# Autodesk Inventor assembly: insertAssembly-2
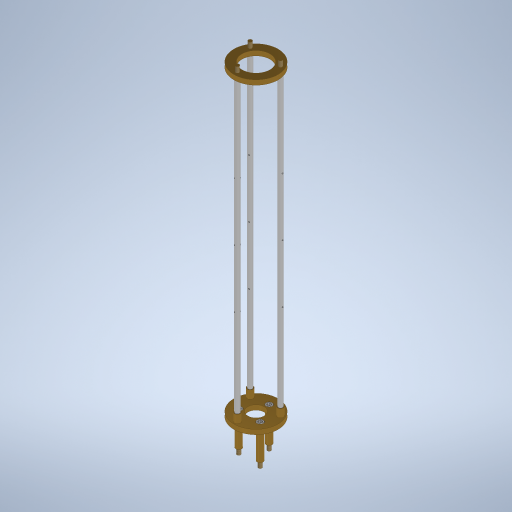
[picture p0: Inventor's stored thumbnail of the model, 512x512]
Saved by Autodesk Inventor 2024 (Build 280153000, 153)
## iProperties
Created: 2023-09-24
Part Number: insertAssembly-2
Document SubType Name: Assembly
Designer: schanen
Author: schanen
## Documents named in this file (6)
- C:\Users\schanen\Documents\Inventor\he4inserts\insertAssembly-2.iam
- C:\Users\schanen\Documents\Inventor\he4inserts\CompositeSupport.iam
- C:\Users\schanen\Documents\Inventor\he4inserts\Insert_flange.ipt
- C:\Users\schanen\Documents\Inventor\he4inserts\Insert_flange_Top.ipt
- C:\Users\schanen\Documents\Inventor\he4inserts\Screw_StainlessSteal_M3_SocketCap_6mm.ipt
- C:\Users\schanen\Documents\Inventor\he4inserts\Fitting-3.ipt
## Components (14 placed, 5 different names)
1. Insert_flange:1 — Mate:9, Mate:10, Mate:11
2. Insert_flange_Top:1 — Mate:5, Mate:6, Mate:7, Mate:8, Mate:12, Mate:13, Mate:14, Mate:15
3. Fitting-3:1 [sub-assembly] — Mate:12, Mate:13
4. Screw_StainlessSteal_M3_SocketCap_6mm:1 — Mate:14, Mate:15
5. Fitting-3:2 [sub-assembly]
6. Screw_StainlessSteal_M3_SocketCap_6mm:2
7. Fitting-3:3 [sub-assembly]
8. Screw_StainlessSteal_M3_SocketCap_6mm:3
9. Screw_StainlessSteal_M3_SocketCap_6mm:4 — Mate:7, Mate:8
10. CompositeSupport:1 [sub-assembly] — Mate:5, Mate:6
11. Screw_StainlessSteal_M3_SocketCap_6mm:5
12. CompositeSupport:2 [sub-assembly] — Mate:10
13. Screw_StainlessSteal_M3_SocketCap_6mm:6
14. CompositeSupport:3 [sub-assembly] — Mate:9, Mate:11
## Component patterns: (3 elements, first: Fitting-3:1 + Screw_StainlessSteal_M3_SocketCap_6mm:1), (3 elements, first: Screw_StainlessSteal_M3_SocketCap_6mm:4 + CompositeSupport:1)
## Relationships (11: Mate 11)
- Mate:5: Insert_flange_Top:1 ↔ CompositeSupport:1
- Mate:6: Insert_flange_Top:1 ↔ CompositeSupport:1
- Mate:7: Insert_flange_Top:1 ↔ Screw_StainlessSteal_M3_SocketCap_6mm:4
- Mate:8: Insert_flange_Top:1 ↔ Screw_StainlessSteal_M3_SocketCap_6mm:4
- Mate:9: Insert_flange:1 ↔ CompositeSupport:3
- Mate:10: Insert_flange:1 ↔ CompositeSupport:2
- Mate:11: Insert_flange:1 ↔ CompositeSupport:3
- Mate:12: Insert_flange_Top:1 ↔ Fitting-3:1
- Mate:13: Insert_flange_Top:1 ↔ Fitting-3:1
- Mate:14: Insert_flange_Top:1 ↔ Screw_StainlessSteal_M3_SocketCap_6mm:1
- Mate:15: Insert_flange_Top:1 ↔ Screw_StainlessSteal_M3_SocketCap_6mm:1
